# Autodesk Inventor assembly: arm
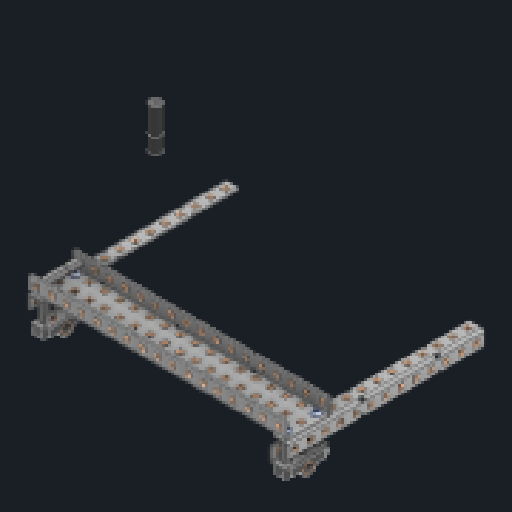
[picture p0: Inventor's stored thumbnail of the model, 512x512]
Saved by Autodesk Inventor 2025 (Build 290162000, 162)
## iProperties
Created: 2024-10-13
Part Number: arm
Document SubType Name: Assembly
Designer: Averey Ku
Author: Averey Ku
## Documents named in this file (12)
- D:\vex_robotics_high_stakes\hardware\cad\bots\high_stakes_v2\intake\arm.iam
- D:\vex_robotics_high_stakes\hardware\cad\robpros_cad_lib\Structure\Angle\Aluminum 1x1\Alu Angle 1x1x13.ipt
- D:\vex_robotics_high_stakes\hardware\cad\robpros_cad_lib\Structure\C Channel\Aluminum 1x3x1\Alu C 1x3x1x17.ipt
- D:\vex_robotics_high_stakes\hardware\cad\robpros_cad_lib\Structure\Angle\Aluminum 1x1\Alu Angle 1x1x3.ipt
- D:\vex_robotics_high_stakes\hardware\cad\robpros_cad_lib\Motion\Shaft HS\HS Pillow Bearing Block.ipt
- D:\vex_robotics_high_stakes\hardware\cad\robpros_cad_lib\Structure\Hardware\Screw Shoulder Robosource.ipt
- D:\vex_robotics_high_stakes\hardware\cad\robpros_cad_lib\Structure\Standoff.ipt
- D:\vex_robotics_high_stakes\hardware\cad\robpros_cad_lib\Structure\Hardware\Screw Shoulder Robosource\SScrew Shoulder Smooth .375 x .12.ipt
- D:\vex_robotics_high_stakes\hardware\cad\robpros_cad_lib\Structure\Standoff\Standoff .75.ipt
- D:\vex_robotics_high_stakes\hardware\cad\robpros_cad_lib\Motion\Spacers\Spacer Nylon .375 OD\NSpacer .375 OD x .500.ipt
- D:\vex_robotics_high_stakes\hardware\cad\robpros_cad_lib\Motion\Spacers\Spacer Nylon .375 OD.ipt
- D:\vex_robotics_high_stakes\hardware\cad\robpros_cad_lib\Motion\Spacers\Spacer Nylon .375 OD\NSpacer .375 OD x .875.ipt
## Components (19 placed, 8 different names)
1. Alu Angle 1x1x13:1 — Mate:4, Angle:1, Insert:3, Mate:5
2. Alu Angle 1x1x13:2 — Insert:4, Mate:6
3. Alu C 1x3x1x17:1 — Insert:19, Insert:20, Insert:21, Insert:22, Insert:28, Insert:30
4. Alu Angle 1x1x3:1 — Insert:4, Mate:6, Insert:6, Mate:8, Insert:23, Insert:24
5. Alu Angle 1x1x3:2 — Insert:3, Mate:5, Insert:5, Mate:7, Insert:25, Insert:26
6. HS Pillow Bearing Block:1 — Insert:5, Mate:7
7. HS Pillow Bearing Block:2 — Insert:6, Mate:8
8. SScrew Shoulder Smooth .375 x .12:3 — Insert:19
9. SScrew Shoulder Smooth .375 x .12:4 — Insert:20
10. SScrew Shoulder Smooth .375 x .12:5 — Insert:22
11. SScrew Shoulder Smooth .375 x .12:6 — Insert:21
12. Standoff .75:5 — Insert:23
13. Standoff .75:6 — Insert:25
14. Standoff .75:7 — Insert:24
15. Standoff .75:8 — Insert:26
16. NSpacer .375 OD x .500:1 — Insert:27
17. NSpacer .375 OD x .875:2 — Insert:27, Insert:28
18. NSpacer .375 OD x .500:3 — Insert:30
19. NSpacer .375 OD x .875:4
## Relationships (27: Insert 18, Mate 8, Angle 1)
- [Mate]: Alu Angle 1x1x13:1 ↔ Alu Angle 1x1x13:2
- [Insert]: Alu Angle 1x1x13:1 ↔ Alu C 1x3x1x17:1
- [Mate]: Alu Angle 1x1x13:1 ↔ Alu C 1x3x1x17:1
- [Insert]: Alu Angle 1x1x13:2 ↔ Alu C 1x3x1x17:1
- [Mate]: Alu Angle 1x1x13:2 ↔ Alu C 1x3x1x17:1
- Mate:4: Alu Angle 1x1x13:1
- Angle:1 (0 deg): Alu Angle 1x1x13:1
- Insert:3 (19.05 mm): Alu Angle 1x1x13:1 ↔ Alu Angle 1x1x3:2
- Mate:5: Alu Angle 1x1x13:1 ↔ Alu Angle 1x1x3:2
- Insert:4 (19.05 mm): Alu Angle 1x1x13:2 ↔ Alu Angle 1x1x3:1
- Mate:6: Alu Angle 1x1x13:2 ↔ Alu Angle 1x1x3:1
- Insert:5: Alu Angle 1x1x3:2 ↔ HS Pillow Bearing Block:1
- Mate:7: Alu Angle 1x1x3:2 ↔ HS Pillow Bearing Block:1
- Insert:6: Alu Angle 1x1x3:1 ↔ HS Pillow Bearing Block:2
- Mate:8: Alu Angle 1x1x3:1 ↔ HS Pillow Bearing Block:2
- Insert:19: Alu C 1x3x1x17:1 ↔ SScrew Shoulder Smooth .375 x .12:3
- Insert:20: Alu C 1x3x1x17:1 ↔ SScrew Shoulder Smooth .375 x .12:4
- Insert:21: Alu C 1x3x1x17:1 ↔ SScrew Shoulder Smooth .375 x .12:6
- Insert:22: Alu C 1x3x1x17:1 ↔ SScrew Shoulder Smooth .375 x .12:5
- Insert:23: Alu Angle 1x1x3:1 ↔ Standoff .75:5
- Insert:24: Alu Angle 1x1x3:1 ↔ Standoff .75:7
- Insert:25: Alu Angle 1x1x3:2 ↔ Standoff .75:6
- Insert:26: Alu Angle 1x1x3:2 ↔ Standoff .75:8
- Insert:27: NSpacer .375 OD x .500:1 ↔ NSpacer .375 OD x .875:2
- Insert:28: Alu C 1x3x1x17:1 ↔ NSpacer .375 OD x .875:2
- [Insert]: NSpacer .375 OD x .500:3 ↔ NSpacer .375 OD x .875:4
- Insert:30: Alu C 1x3x1x17:1 ↔ NSpacer .375 OD x .500:3
## Named parameters: d44_d42 = 0 mm
